# Autodesk Inventor assembly: MG_996R
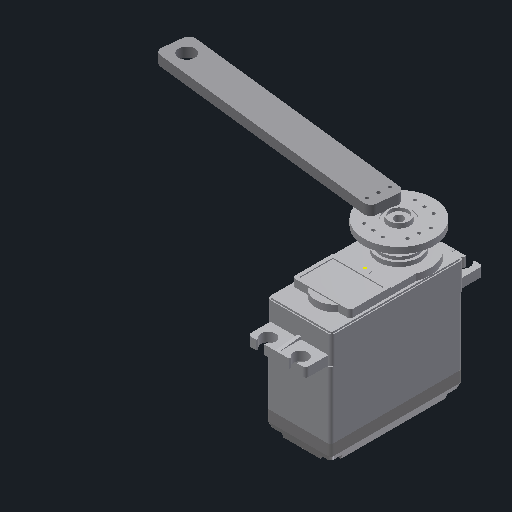
[picture p0: Inventor's stored thumbnail of the model, 512x512]
Saved by Autodesk Inventor 2023.6 (Build 276521000, 521)
## iProperties
Created: 2016-09-26
Part Number: MG_996R
Document SubType Name: Assembly
Designer: Julian
Author: Julian
## Documents named in this file (7)
- D:\FP (Sebelum Revisi)\MG_996R.iam
- D:\FP (Sebelum Revisi)\Base.ipt
- D:\FP (Sebelum Revisi)\Medio.ipt
- D:\FP (Sebelum Revisi)\Top.ipt
- D:\FP (Sebelum Revisi)\Eje.ipt
- D:\FP (Sebelum Revisi)\Acople circular.ipt
- D:\FP (Sebelum Revisi)\FP V2 Servo Arm.ipt
## Components (6 placed, 6 different names)
1. Top:1 — Rígido:2, De rotación:1
2. Medio:1 — Rígido:1, Rígido:2
3. Base:1 — Rígido:1
4. Eje:1 — De rotación:1, Mate:1, Mate:2
5. Acople circular:1 — Mate:1, Mate:2, Mate:3, Mate:4, Mate:5, Mate:6
6. FP V2 Servo Arm:1 — Mate:3, Mate:4, Mate:5, Mate:6
## Relationships (9: Mate 6, WeldJoint 2, RevoluteJoint 1)
- Rígido:1 [WeldJoint]: Medio:1 ↔ Base:1
- Rígido:2 [WeldJoint]: Top:1 ↔ Medio:1
- De rotación:1 [RevoluteJoint]: Top:1 ↔ Eje:1
- Mate:1: Eje:1 ↔ Acople circular:1
- Mate:2: Eje:1 ↔ Acople circular:1
- Mate:3: Acople circular:1 ↔ FP V2 Servo Arm:1
- Mate:4: Acople circular:1 ↔ FP V2 Servo Arm:1
- Mate:5: Acople circular:1 ↔ FP V2 Servo Arm:1
- Mate:6: Acople circular:1 ↔ FP V2 Servo Arm:1
